# Autodesk Inventor assembly: CORL_000_CoralAssembly
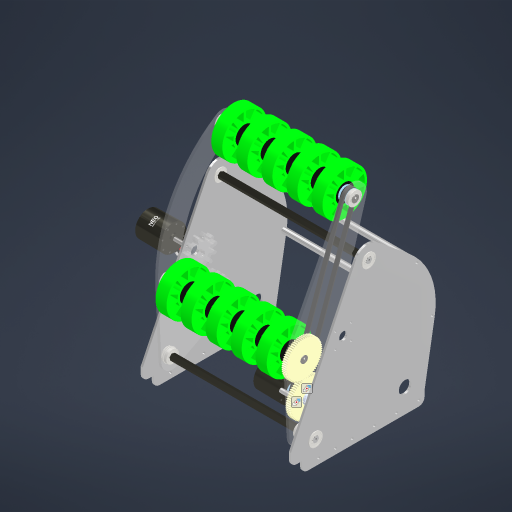
[picture p0: Inventor's stored thumbnail of the model, 512x512]
Saved by Autodesk Inventor 2024.2 (Build 282272000, 272)
## iProperties
Created: 2024-08-02
Part Number: CORL_000_CoralAssembly
Document SubType Name: Assembly
Designer: Bryan
Mass: 1860.11 g
Surface Area: 4686.68 cm^2
Volume: 1141.27 cm^3
Density: 1.62986 g/cm^3
Author: Bryan
## Documents named in this file (21)
- C:\Users\bobsb\OneDrive\Documents\GitHub\1622-2024-Summer-CAD-A-Thon\Coral\CORL_000_CoralAssembly.iam
- C:\Users\bobsb\OneDrive\Documents\GitHub\1622-2024-Summer-CAD-A-Thon\Coral\CORL_001_MainPlate.ipt
- C:\Users\bobsb\OneDrive\Documents\GitHub\1622-2024-Summer-CAD-A-Thon\COTS Library\Motion\Bearings\COTS_WCP-0783_1.125ODHexBearing.ipt
- C:\Users\bobsb\OneDrive\Documents\GitHub\1622-2024-Summer-CAD-A-Thon\Coral\CORL_002_FanPlate.ipt
- C:\Users\bobsb\OneDrive\Documents\GitHub\1622-2024-Summer-CAD-A-Thon\Coral\CORL_003_DropShaft.ipt
- C:\Users\bobsb\OneDrive\Documents\GitHub\1622-2024-Summer-CAD-A-Thon\Coral\CORL_004_PivotShaft.ipt
- C:\Users\bobsb\OneDrive\Documents\GitHub\1622-2024-Summer-CAD-A-Thon\Coral\CORL_005_PolyCarbSprocket.ipt
- C:\Users\bobsb\OneDrive\Documents\GitHub\1622-2024-Summer-CAD-A-Thon\Coral\CORL_006_SmallPlate.ipt
- C:\Users\bobsb\OneDrive\Documents\GitHub\1622-2024-Summer-CAD-A-Thon\COTS Library\Motors\COTS_REV-21-1650-V1.1.ipt
- C:\Users\bobsb\OneDrive\Documents\GitHub\1622-2024-Summer-CAD-A-Thon\Coral\CORL_009_LongStandoff.ipt
- C:\Users\bobsb\OneDrive\Documents\GitHub\1622-2024-Summer-CAD-A-Thon\COTS Library\Adapters\COTS_REV-21-1879_8mmKeyTo0.5Hex.ipt
- C:\Users\bobsb\OneDrive\Documents\GitHub\1622-2024-Summer-CAD-A-Thon\COTS Library\Motion\Gears\20DP gears\Aluminum\COTS_WCP-0722.ipt
- C:\Users\bobsb\OneDrive\Documents\GitHub\1622-2024-Summer-CAD-A-Thon\COTS Library\Motion\Pulleys\HTD5M\10mm Wide\COTS_HTD5MM_10mm_20T.ipt
- C:\Users\bobsb\OneDrive\Documents\GitHub\1622-2024-Summer-CAD-A-Thon\COTS Library\Fasteners\Bolts\Button-Head\10-32\COTS_91255A275_1.5in long Button Head Hex Drive Screw.ipt
- C:\Users\bobsb\OneDrive\Documents\GitHub\1622-2024-Summer-CAD-A-Thon\COTS Library\Fasteners\Bolts\Button-Head\10-32\COTS_92949A265_1-2in long Stainless Steel Button Head Screw.ipt
- C:\Users\bobsb\OneDrive\Documents\GitHub\1622-2024-Summer-CAD-A-Thon\COTS Library\Fasteners\Shaft Collars\COTS_WCP-0799_0.5inchHexShaftCollar.ipt
- C:\Users\bobsb\OneDrive\Documents\GitHub\1622-2024-Summer-CAD-A-Thon\COTS Library\Fasteners\Washers\COTS_90107A029_316 Stainless Steel Washer.ipt
- C:\Users\bobsb\OneDrive\Documents\GitHub\1622-2024-Summer-CAD-A-Thon\Coral\CORL_010_DropGearShaft.ipt
- C:\Users\bobsb\OneDrive\Documents\GitHub\1622-2024-Summer-CAD-A-Thon\COTS Library\Motion\Wheels\Compliant Wheels\4in compliant wheels\0.500in hex bore\COTS_am-3462_4indiameter_0.500inhexbore_durometer35A_CompliantWheel.ipt
- C:\Users\bobsb\OneDrive\Documents\GitHub\1622-2024-Summer-CAD-A-Thon\Coral\CORL_011_NEOStandoff.ipt
- C:\Users\bobsb\OneDrive\Documents\GitHub\1622-2024-Summer-CAD-A-Thon\Coral\CORL_012_ArmBelt.ipt
## Components (56 placed, 20 different names)
1. CORL_001_MainPlate:1 — Mate:3, Mate:7, Mate:18, Mate:26, Mate:72, Mate:75, Mate:76, Mate:77, Mate:81, Mate:83, Mate:84, Mate:85, Flush:17
2. CORL_001_MainPlate:2 — Mate:3, Mate:10, Mate:29, Mate:47, Mate:67, Mate:68, Mate:76, Mate:77, Mate:79, Mate:80
3. COTS_WCP-0783_1.125ODHexBearing:2 — Mate:70, Flush:16, Mate:75, Mate:81
4. COTS_WCP-0783_1.125ODHexBearing:4 — Mate:7, Mate:26, Mate:30, Flush:2, Mate:78
5. COTS_WCP-0783_1.125ODHexBearing:7 — Mate:10, Mate:29
6. COTS_WCP-0783_1.125ODHexBearing:10 — Mate:79, Mate:80
7. CORL_002_FanPlate:2 — Mate:18, Mate:23, Mate:27, Flush:13, Mate:78, Mate:82, Mate:86, Mate:87, Mate:125, Mate:126
8. COTS_WCP-0783_1.125ODHexBearing:11 — Mate:27, Mate:82
9. COTS_WCP-0783_1.125ODHexBearing:12 — Mate:33, Flush:5, Mate:36, Mate:37
10. COTS_WCP-0783_1.125ODHexBearing:13 — Flush:5, Mate:35
11. COTS_WCP-0783_1.125ODHexBearing:14 — Mate:23, Mate:86, Mate:119, Flush:21
12. CORL_004_PivotShaft:1 — Mate:30, Flush:2, Mate:33
13. CORL_006_SmallPlate:1 — Mate:35, Mate:36, Mate:37, Mate:47, Mate:88, Mate:95, Mate:96, Mate:97, Mate:102, Mate:104, Mate:105, Mate:106, Mate:107, Mate:108, Mate:109, Mate:110, Mate:111
14. CORL_005_PolyCarbSprocket:3 — Mate:58, Mate:59, Mate:60
15. CORL_005_PolyCarbSprocket:4 — Mate:58, Mate:59, Mate:60, Flush:13, Mate:72
16. CORL_009_LongStandoff:1 — Mate:67, Mate:84
17. CORL_009_LongStandoff:2 — Mate:68, Mate:83
18. CORL_004_PivotShaft:3 — Mate:70, Flush:16
19. COTS_REV-21-1650-V1.1:1 — Mate:85
20. CORL_003_DropShaft:2 — Mate:87, Mate:103, Flush:20, Mate:142, Mate:143
21. COTS_REV-21-1650-V1.1:2 — Mate:88, Mate:89, Mate:90, Mate:91, Mate:92, Mate:93, Mate:99, Mate:102, Mate:113, Mate:133, Mate:134, Mate:135, Mate:136
22. COTS_REV-21-1879_8mmKeyTo0.5Hex:1 — Mate:89, Mate:90, Mate:100
23. COTS_WCP-0722:1 — Mate:91, Mate:101, Mate:112, Mate:115
24. COTS_HTD5MM_10mm_20T:1 — Mate:92, Mate:93, Flush:19, Mate:139
25. COTS_HTD5MM_10mm_20T:2 — Mate:95, Flush:19, Mate:98, Mate:137, Mate:138, Mate:144
26. COTS_WCP-0783_1.125ODHexBearing:15 — Mate:96, Mate:97, Mate:98, Mate:103, Flush:20
27. COTS_REV-21-1879_8mmKeyTo0.5Hex:2 — Mate:99, Mate:100, Mate:101, Mate:114, Mate:116
28. COTS_91255A275_1.5in long Button Head Hex Drive Screw:1 — Mate:104, Mate:105, Mate:129
29. COTS_91255A275_1.5in long Button Head Hex Drive Screw:2 — Mate:106, Mate:109, Mate:112, Mate:130
30. COTS_91255A275_1.5in long Button Head Hex Drive Screw:3 — Mate:107, Mate:110, Mate:131
31. COTS_91255A275_1.5in long Button Head Hex Drive Screw:4 — Mate:108, Mate:111, Mate:132
32. COTS_92949A265_1-2in long Stainless Steel Button Head Screw:1 — Mate:113, Mate:118
33. COTS_WCP-0799_0.5inchHexShaftCollar:1 — Mate:114, Mate:115, Mate:117
34. COTS_90107A029_316 Stainless Steel Washer:1 — Mate:116, Mate:117, Mate:118
35. CORL_010_DropGearShaft:1 — Mate:119, Flush:21, Flush:22, Mate:120, Mate:122, Mate:124, Mate:127
36. COTS_WCP-0722:2 — Flush:22, Mate:120
37. COTS_92949A265_1-2in long Stainless Steel Button Head Screw:2 — Mate:122, Mate:123
38. COTS_90107A029_316 Stainless Steel Washer:2 — Mate:123, Mate:124
39. COTS_WCP-0783_1.125ODHexBearing:16 — Mate:125, Mate:126
40. CORL_011_NEOStandoff:1 — Mate:129, Mate:134
41. CORL_011_NEOStandoff:2 — Mate:130, Mate:135
42. CORL_011_NEOStandoff:3 — Mate:132, Mate:136
43. CORL_011_NEOStandoff:4 — Mate:131, Mate:133
44. CORL_012_ArmBelt:1 — Mate:137, Mate:138, Mate:139
45. COTS_92949A265_1-2in long Stainless Steel Button Head Screw:3 — Mate:142
46. COTS_90107A029_316 Stainless Steel Washer:3 — Mate:143
47. COTS_am-3462_4indiameter_0.500inhexbore_durometer35A_CompliantWheel:1 — Mate:127, Tangent:1
48. COTS_am-3462_4indiameter_0.500inhexbore_durometer35A_CompliantWheel:2
49. COTS_am-3462_4indiameter_0.500inhexbore_durometer35A_CompliantWheel:3
50. COTS_am-3462_4indiameter_0.500inhexbore_durometer35A_CompliantWheel:4
51. COTS_am-3462_4indiameter_0.500inhexbore_durometer35A_CompliantWheel:5
52. COTS_am-3462_4indiameter_0.500inhexbore_durometer35A_CompliantWheel:6
53. COTS_am-3462_4indiameter_0.500inhexbore_durometer35A_CompliantWheel:7
54. COTS_am-3462_4indiameter_0.500inhexbore_durometer35A_CompliantWheel:8
55. COTS_am-3462_4indiameter_0.500inhexbore_durometer35A_CompliantWheel:9
56. COTS_am-3462_4indiameter_0.500inhexbore_durometer35A_CompliantWheel:10 — Mate:144
## Component patterns: (10 elements, first: COTS_am-3462_4indiameter_0.500inhexbore_durometer35A_CompliantWheel:1)
## Relationships (99: Mate 89, Flush 9, Tangent 1)
- Mate:3 (333.375 mm): CORL_001_MainPlate:1 ↔ CORL_001_MainPlate:2
- Mate:7: CORL_001_MainPlate:1 ↔ COTS_WCP-0783_1.125ODHexBearing:4
- Mate:10: CORL_001_MainPlate:2 ↔ COTS_WCP-0783_1.125ODHexBearing:7
- Mate:18 (6.35 mm): CORL_001_MainPlate:1 ↔ CORL_002_FanPlate:2
- Mate:23: CORL_002_FanPlate:2 ↔ COTS_WCP-0783_1.125ODHexBearing:14
- Mate:26: CORL_001_MainPlate:1 ↔ COTS_WCP-0783_1.125ODHexBearing:4
- Mate:27: CORL_002_FanPlate:2 ↔ COTS_WCP-0783_1.125ODHexBearing:11
- Mate:29: CORL_001_MainPlate:2 ↔ COTS_WCP-0783_1.125ODHexBearing:7
- Mate:30: COTS_WCP-0783_1.125ODHexBearing:4 ↔ CORL_004_PivotShaft:1
- Flush:2: COTS_WCP-0783_1.125ODHexBearing:4 ↔ CORL_004_PivotShaft:1
- Mate:33: COTS_WCP-0783_1.125ODHexBearing:12 ↔ CORL_004_PivotShaft:1
- Flush:5: COTS_WCP-0783_1.125ODHexBearing:12 ↔ COTS_WCP-0783_1.125ODHexBearing:13
- Mate:35: COTS_WCP-0783_1.125ODHexBearing:13 ↔ CORL_006_SmallPlate:1
- Mate:36: COTS_WCP-0783_1.125ODHexBearing:12 ↔ CORL_006_SmallPlate:1
- Mate:37: COTS_WCP-0783_1.125ODHexBearing:12 ↔ CORL_006_SmallPlate:1
- Mate:47 (25.4 mm): CORL_001_MainPlate:2 ↔ CORL_006_SmallPlate:1
- Mate:58: CORL_005_PolyCarbSprocket:3 ↔ CORL_005_PolyCarbSprocket:4
- Mate:59: CORL_005_PolyCarbSprocket:3 ↔ CORL_005_PolyCarbSprocket:4
- Mate:60: CORL_005_PolyCarbSprocket:3 ↔ CORL_005_PolyCarbSprocket:4
- Flush:13 (-3.175 mm): CORL_002_FanPlate:2 ↔ CORL_005_PolyCarbSprocket:4
- Mate:67: CORL_001_MainPlate:2 ↔ CORL_009_LongStandoff:1
- Mate:68: CORL_001_MainPlate:2 ↔ CORL_009_LongStandoff:2
- Mate:70: COTS_WCP-0783_1.125ODHexBearing:2 ↔ CORL_004_PivotShaft:3
- Flush:16: COTS_WCP-0783_1.125ODHexBearing:2 ↔ CORL_004_PivotShaft:3
- Mate:72: CORL_001_MainPlate:1 ↔ CORL_005_PolyCarbSprocket:4
- Mate:75: CORL_001_MainPlate:1 ↔ COTS_WCP-0783_1.125ODHexBearing:2
- Mate:76: CORL_001_MainPlate:1 ↔ CORL_001_MainPlate:2
- Mate:77: CORL_001_MainPlate:1 ↔ CORL_001_MainPlate:2
- Mate:78: COTS_WCP-0783_1.125ODHexBearing:4 ↔ CORL_002_FanPlate:2
- Mate:79: CORL_001_MainPlate:2 ↔ COTS_WCP-0783_1.125ODHexBearing:10
- Mate:80: CORL_001_MainPlate:2 ↔ COTS_WCP-0783_1.125ODHexBearing:10
- Mate:81: CORL_001_MainPlate:1 ↔ COTS_WCP-0783_1.125ODHexBearing:2
- Mate:82: CORL_002_FanPlate:2 ↔ COTS_WCP-0783_1.125ODHexBearing:11
- Mate:83: CORL_001_MainPlate:1 ↔ CORL_009_LongStandoff:2
- Mate:84: CORL_001_MainPlate:1 ↔ CORL_009_LongStandoff:1
- Mate:85: CORL_001_MainPlate:1 ↔ COTS_REV-21-1650-V1.1:1
- Mate:86: CORL_002_FanPlate:2 ↔ COTS_WCP-0783_1.125ODHexBearing:14
- Flush:17 (28.575 mm): CORL_001_MainPlate:1
- Mate:87: CORL_002_FanPlate:2 ↔ CORL_003_DropShaft:2
- Mate:88: CORL_006_SmallPlate:1 ↔ COTS_REV-21-1650-V1.1:2
- Mate:89: COTS_REV-21-1650-V1.1:2 ↔ COTS_REV-21-1879_8mmKeyTo0.5Hex:1
- Mate:90: COTS_REV-21-1650-V1.1:2 ↔ COTS_REV-21-1879_8mmKeyTo0.5Hex:1
- Mate:91: COTS_REV-21-1650-V1.1:2 ↔ COTS_WCP-0722:1
- Mate:92: COTS_REV-21-1650-V1.1:2 ↔ COTS_HTD5MM_10mm_20T:1
- Mate:93: COTS_REV-21-1650-V1.1:2 ↔ COTS_HTD5MM_10mm_20T:1
- Mate:95: CORL_006_SmallPlate:1 ↔ COTS_HTD5MM_10mm_20T:2
- Flush:19: COTS_HTD5MM_10mm_20T:1 ↔ COTS_HTD5MM_10mm_20T:2
- Mate:96: CORL_006_SmallPlate:1 ↔ COTS_WCP-0783_1.125ODHexBearing:15
- Mate:97: CORL_006_SmallPlate:1 ↔ COTS_WCP-0783_1.125ODHexBearing:15
- Mate:98: COTS_HTD5MM_10mm_20T:2 ↔ COTS_WCP-0783_1.125ODHexBearing:15
- Mate:99: COTS_REV-21-1650-V1.1:2 ↔ COTS_REV-21-1879_8mmKeyTo0.5Hex:2
- Mate:100: COTS_REV-21-1879_8mmKeyTo0.5Hex:1 ↔ COTS_REV-21-1879_8mmKeyTo0.5Hex:2
- Mate:101: COTS_WCP-0722:1 ↔ COTS_REV-21-1879_8mmKeyTo0.5Hex:2
- Mate:102: CORL_006_SmallPlate:1 ↔ COTS_REV-21-1650-V1.1:2
- Mate:103: CORL_003_DropShaft:2 ↔ COTS_WCP-0783_1.125ODHexBearing:15
- Flush:20: CORL_003_DropShaft:2 ↔ COTS_WCP-0783_1.125ODHexBearing:15
- Mate:104: CORL_006_SmallPlate:1 ↔ COTS_91255A275_1.5in long Button Head Hex Drive Screw:1
- Mate:105: CORL_006_SmallPlate:1 ↔ COTS_91255A275_1.5in long Button Head Hex Drive Screw:1
- Mate:106: CORL_006_SmallPlate:1 ↔ COTS_91255A275_1.5in long Button Head Hex Drive Screw:2
- Mate:107: CORL_006_SmallPlate:1 ↔ COTS_91255A275_1.5in long Button Head Hex Drive Screw:3
- Mate:108: CORL_006_SmallPlate:1 ↔ COTS_91255A275_1.5in long Button Head Hex Drive Screw:4
- Mate:109: CORL_006_SmallPlate:1 ↔ COTS_91255A275_1.5in long Button Head Hex Drive Screw:2
- Mate:110: CORL_006_SmallPlate:1 ↔ COTS_91255A275_1.5in long Button Head Hex Drive Screw:3
- Mate:111: CORL_006_SmallPlate:1 ↔ COTS_91255A275_1.5in long Button Head Hex Drive Screw:4
- Mate:112: COTS_WCP-0722:1 ↔ COTS_91255A275_1.5in long Button Head Hex Drive Screw:2
- Mate:113: COTS_REV-21-1650-V1.1:2 ↔ COTS_92949A265_1-2in long Stainless Steel Button Head Screw:1
- Mate:114: COTS_REV-21-1879_8mmKeyTo0.5Hex:2 ↔ COTS_WCP-0799_0.5inchHexShaftCollar:1
- Mate:115: COTS_WCP-0722:1 ↔ COTS_WCP-0799_0.5inchHexShaftCollar:1
- Mate:116: COTS_REV-21-1879_8mmKeyTo0.5Hex:2 ↔ COTS_90107A029_316 Stainless Steel Washer:1
- Mate:117: COTS_WCP-0799_0.5inchHexShaftCollar:1 ↔ COTS_90107A029_316 Stainless Steel Washer:1
- Mate:118: COTS_92949A265_1-2in long Stainless Steel Button Head Screw:1 ↔ COTS_90107A029_316 Stainless Steel Washer:1
- Mate:119: COTS_WCP-0783_1.125ODHexBearing:14 ↔ CORL_010_DropGearShaft:1
- Flush:21: COTS_WCP-0783_1.125ODHexBearing:14 ↔ CORL_010_DropGearShaft:1
- Flush:22: CORL_010_DropGearShaft:1 ↔ COTS_WCP-0722:2
- Mate:120: CORL_010_DropGearShaft:1 ↔ COTS_WCP-0722:2
- [Mate]: COTS_92949A265_1-2in long Stainless Steel Button Head Screw:2 ↔ COTS_90107A029_316 Stainless Steel Washer:2
- Mate:122: CORL_010_DropGearShaft:1 ↔ COTS_92949A265_1-2in long Stainless Steel Button Head Screw:2
- Mate:123: COTS_92949A265_1-2in long Stainless Steel Button Head Screw:2 ↔ COTS_90107A029_316 Stainless Steel Washer:2
- Mate:124: CORL_010_DropGearShaft:1 ↔ COTS_90107A029_316 Stainless Steel Washer:2
- Mate:125: CORL_002_FanPlate:2 ↔ COTS_WCP-0783_1.125ODHexBearing:16
- Mate:126: CORL_002_FanPlate:2 ↔ COTS_WCP-0783_1.125ODHexBearing:16
- Mate:127: CORL_010_DropGearShaft:1 ↔ COTS_am-3462_4indiameter_0.500inhexbore_durometer35A_CompliantWheel:1
- Mate:129: COTS_91255A275_1.5in long Button Head Hex Drive Screw:1 ↔ CORL_011_NEOStandoff:1
- Mate:130: COTS_91255A275_1.5in long Button Head Hex Drive Screw:2 ↔ CORL_011_NEOStandoff:2
- Mate:131: COTS_91255A275_1.5in long Button Head Hex Drive Screw:3 ↔ CORL_011_NEOStandoff:4
- Mate:132: COTS_91255A275_1.5in long Button Head Hex Drive Screw:4 ↔ CORL_011_NEOStandoff:3
- Mate:133: COTS_REV-21-1650-V1.1:2 ↔ CORL_011_NEOStandoff:4
- Mate:134: COTS_REV-21-1650-V1.1:2 ↔ CORL_011_NEOStandoff:1
- Mate:135: COTS_REV-21-1650-V1.1:2 ↔ CORL_011_NEOStandoff:2
- Mate:136: COTS_REV-21-1650-V1.1:2 ↔ CORL_011_NEOStandoff:3
- Mate:137: COTS_HTD5MM_10mm_20T:2 ↔ CORL_012_ArmBelt:1
- Mate:138: COTS_HTD5MM_10mm_20T:2 ↔ CORL_012_ArmBelt:1
- Mate:139: COTS_HTD5MM_10mm_20T:1 ↔ CORL_012_ArmBelt:1
- [Mate]: COTS_92949A265_1-2in long Stainless Steel Button Head Screw:3 ↔ COTS_90107A029_316 Stainless Steel Washer:3
- [Mate]: COTS_92949A265_1-2in long Stainless Steel Button Head Screw:3 ↔ COTS_90107A029_316 Stainless Steel Washer:3
- Mate:142: CORL_003_DropShaft:2 ↔ COTS_92949A265_1-2in long Stainless Steel Button Head Screw:3
- Mate:143: CORL_003_DropShaft:2 ↔ COTS_90107A029_316 Stainless Steel Washer:3
- Tangent:1: COTS_am-3462_4indiameter_0.500inhexbore_durometer35A_CompliantWheel:1
- Mate:144: COTS_HTD5MM_10mm_20T:2 ↔ COTS_am-3462_4indiameter_0.500inhexbore_durometer35A_CompliantWheel:10
## Named parameters: d173_d168 = 0 mm, d196_d173_d168 = 0 mm, d197_d175 = 0 mm
